# Autodesk Inventor assembly: Chassis-SubAssem01
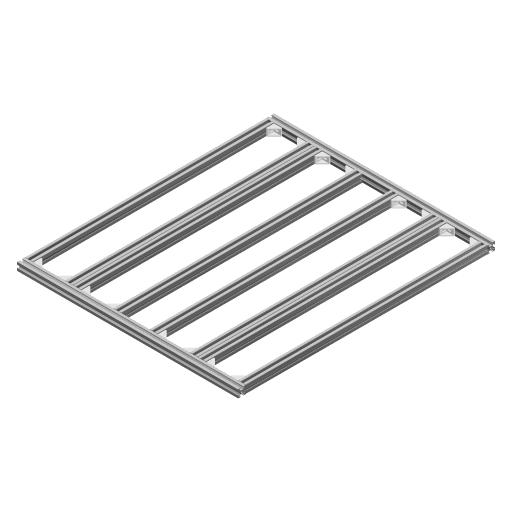
[picture p0: Inventor's stored thumbnail of the model, 512x512]
Saved by Autodesk Inventor 2024.1 (Build 281209000, 209)
## iProperties
Created: 2023-10-26
Part Number: Chassis-SubAssem01
Document SubType Name: Assembly
Designer: david
Author: david
## Documents named in this file (6)
- E:\ChalkbotMechanical\Chalkbot1.0\Chassis\V1\Chassis-SubAssem01.iam
- E:\ChalkbotMechanical\Chalkbot1.0\Chassis\V1\20x20 Channel\20x20 Channel-550.ipt
- C:\Autodesk\ChalkBot Github\ChalkbotMechanical\Chalkbot1.0\Chassis\V1\20x20 Channel.ipt
- E:\ChalkbotMechanical\Chalkbot1.0\Chassis\V1\20x20 Channel\20x20 Channel-600.ipt
- E:\ChalkbotMechanical\Chalkbot1.0\Chassis\V1\20x20 90 Gusset.ipt
- E:\ChalkbotMechanical\Chalkbot1.0\Chassis\V1\20x20 90 Gusset_MIR1.ipt
## Components (26 placed, 4 different names)
1. 20x20 Channel-550:1 — Mate:28, Flush:18, Flush:19
2. 20x20 Channel-550:2 — Mate:1, Flush:1, Mate:3, Flush:3, Flush:4, Mate:5, Flush:5, Mate:7, Flush:6, Mate:9, Mate:11, Flush:7, Flush:9, Mate:12, Flush:10, Mate:15, Mate:17, Flush:11, Flush:12, Mate:18, Flush:13, Mate:21, Flush:14, Mate:22, Mate:24, Flush:15, Mate:27, Flush:16
3. 20x20 Channel-600:3 — Mate:13, Flush:10, Mate:15, Mate:26, Flush:17, Mate:28, Flush:18, Flush:19
4. 20x20 Channel-600:4 — Rigid:2, Flush:9, Mate:12, Mate:14, Mate:23
5. 20x20 Channel-600:5 — Rigid:2, Mate:13, Mate:25
6. 20x20 Channel-600:6 — Mate:10, Mate:11, Flush:7, Mate:14, Mate:20
7. 20x20 Channel-600:7 — Mate:8, Flush:6, Mate:9, Mate:10, Mate:19
8. 20x20 Channel-600:8 — Rigid:1, Flush:4, Mate:8, Mate:16
9. 20x20 Channel-600:9 — Rigid:1, Mate:4, Mate:5, Mate:6
10. 20x20 Channel-600:10 — Mate:2, Flush:2, Mate:3, Flush:3, Mate:4
11. 20x20 90 Gusset:1 — Mate:26, Mate:27, Flush:16
12. 20x20 90 Gusset:6 — Flush:5, Mate:6, Mate:7
13. 20x20 90 Gusset:7 — Flush:12, Mate:18, Mate:19
14. 20x20 90 Gusset:8 — Flush:14, Mate:22, Mate:23
15. 20x20 90 Gusset:9 — Mate:1, Flush:1, Mate:2, Flush:2
16. 20x20 90 Gusset:10 — Mate:16, Mate:17, Flush:11
17. 20x20 90 Gusset:11 — Mate:20, Flush:13, Mate:21
18. 20x20 90 Gusset:12 — Mate:24, Flush:15, Mate:25
19. 20x20 90 Gusset_MIR1:1
20. 20x20 90 Gusset_MIR1:2
21. 20x20 90 Gusset_MIR1:3
22. 20x20 90 Gusset_MIR1:4
23. 20x20 90 Gusset_MIR1:5
24. 20x20 90 Gusset_MIR1:6
25. 20x20 90 Gusset_MIR1:7
26. 20x20 90 Gusset_MIR1:8
## Relationships (48: Mate 28, Flush 18, WeldJoint 2)
- Rigid:1 [WeldJoint]: 20x20 Channel-600:8 ↔ 20x20 Channel-600:9
- Rigid:2 [WeldJoint]: 20x20 Channel-600:4 ↔ 20x20 Channel-600:5
- Mate:1: 20x20 Channel-550:2 ↔ 20x20 90 Gusset:9
- Flush:1 (1.5 mm): 20x20 Channel-550:2 ↔ 20x20 90 Gusset:9
- Mate:2: 20x20 Channel-600:10 ↔ 20x20 90 Gusset:9
- Flush:2 (1.5 mm): 20x20 Channel-600:10 ↔ 20x20 90 Gusset:9
- Mate:3: 20x20 Channel-550:2 ↔ 20x20 Channel-600:10
- Flush:3: 20x20 Channel-550:2 ↔ 20x20 Channel-600:10
- Mate:4 (80 mm): 20x20 Channel-600:9 ↔ 20x20 Channel-600:10
- Flush:4: 20x20 Channel-550:2 ↔ 20x20 Channel-600:8
- Mate:5: 20x20 Channel-550:2 ↔ 20x20 Channel-600:9
- Flush:5 (1.5 mm): 20x20 Channel-550:2 ↔ 20x20 90 Gusset:6
- Mate:6: 20x20 Channel-600:9 ↔ 20x20 90 Gusset:6
- Mate:7: 20x20 Channel-550:2 ↔ 20x20 90 Gusset:6
- Mate:8 (80 mm): 20x20 Channel-600:7 ↔ 20x20 Channel-600:8
- Flush:6: 20x20 Channel-550:2 ↔ 20x20 Channel-600:7
- Mate:9: 20x20 Channel-550:2 ↔ 20x20 Channel-600:7
- Mate:10 (70 mm): 20x20 Channel-600:6 ↔ 20x20 Channel-600:7
- Mate:11: 20x20 Channel-550:2 ↔ 20x20 Channel-600:6
- Flush:7: 20x20 Channel-550:2 ↔ 20x20 Channel-600:6
- Flush:9: 20x20 Channel-550:2 ↔ 20x20 Channel-600:4
- Mate:12: 20x20 Channel-550:2 ↔ 20x20 Channel-600:4
- Mate:13 (80 mm): 20x20 Channel-600:3 ↔ 20x20 Channel-600:5
- Mate:14 (80 mm): 20x20 Channel-600:4 ↔ 20x20 Channel-600:6
- Flush:10: 20x20 Channel-550:2 ↔ 20x20 Channel-600:3
- Mate:15: 20x20 Channel-550:2 ↔ 20x20 Channel-600:3
- Mate:16: 20x20 Channel-600:8 ↔ 20x20 90 Gusset:10
- Mate:17: 20x20 Channel-550:2 ↔ 20x20 90 Gusset:10
- Flush:11 (-1.5 mm): 20x20 Channel-550:2 ↔ 20x20 90 Gusset:10
- Flush:12 (1.5 mm): 20x20 Channel-550:2 ↔ 20x20 90 Gusset:7
- Mate:18: 20x20 Channel-550:2 ↔ 20x20 90 Gusset:7
- Mate:19: 20x20 Channel-600:7 ↔ 20x20 90 Gusset:7
- Mate:20: 20x20 Channel-600:6 ↔ 20x20 90 Gusset:11
- Flush:13 (1.5 mm): 20x20 Channel-550:2 ↔ 20x20 90 Gusset:11
- Mate:21: 20x20 Channel-550:2 ↔ 20x20 90 Gusset:11
- Flush:14 (1.5 mm): 20x20 Channel-550:2 ↔ 20x20 90 Gusset:8
- Mate:22: 20x20 Channel-550:2 ↔ 20x20 90 Gusset:8
- Mate:23: 20x20 Channel-600:4 ↔ 20x20 90 Gusset:8
- Mate:24: 20x20 Channel-550:2 ↔ 20x20 90 Gusset:12
- Flush:15 (-1.5 mm): 20x20 Channel-550:2 ↔ 20x20 90 Gusset:12
- Mate:25: 20x20 Channel-600:5 ↔ 20x20 90 Gusset:12
- Mate:26: 20x20 Channel-600:3 ↔ 20x20 90 Gusset:1
- Mate:27: 20x20 Channel-550:2 ↔ 20x20 90 Gusset:1
- Flush:16 (1.5 mm): 20x20 Channel-550:2 ↔ 20x20 90 Gusset:1
- Flush:17 (-300 mm): 20x20 Channel-600:3
- Mate:28: 20x20 Channel-550:1 ↔ 20x20 Channel-600:3
- Flush:18: 20x20 Channel-550:1 ↔ 20x20 Channel-600:3
- Flush:19: 20x20 Channel-550:1 ↔ 20x20 Channel-600:3
